# Autodesk Inventor assembly: yaw_unit
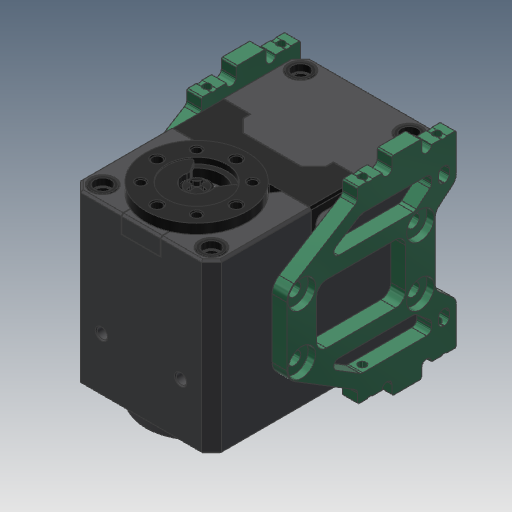
[picture p0: Inventor's stored thumbnail of the model, 512x512]
Saved by Autodesk Inventor 2019.4 (Build 234330000, 330)
## iProperties
Created: 2018-08-06
Part Number: yaw_unit
Material: 一般
Document SubType Name: Assembly
Designer: student
Mass: 66.6076 g
Surface Area: 177.769 cm^2
Volume: 47.0989 cm^3
Density: 1.41421 g/cm^3
Author: student
## Documents named in this file (4)
- C:\Workspace\HaptHexa\Hardware\Inventor\Thorax\yaw_unit\yaw_unit.iam
- C:\Workspace\HaptHexa\Hardware\Inventor\X430\XL-430.iam
- C:\Workspace\HaptHexa\Hardware\Inventor\Thorax\yaw_unit\yaw_servo_side.ipt
- C:\Workspace\HaptHexa\Hardware\Inventor\Thorax\yaw_unit\yaw_servo_side_mir1.ipt
## Components (3 placed, 3 different names)
1. XL-430:1 [sub-assembly] — メイト:1, メイト:2, メイト:3, フラッシュ:1, メイト:4, フラッシュ:2
2. yaw_servo_side:1 — メイト:1, メイト:2, メイト:3
3. yaw_servo_side_mir1:1
## Relationships (6: Mate 4, Flush 2)
- メイト:1 [Mate]: XL-430:1 ↔ yaw_servo_side:1
- メイト:2 [Mate]: XL-430:1 ↔ yaw_servo_side:1
- メイト:3 [Mate]: XL-430:1 ↔ yaw_servo_side:1
- フラッシュ:1 [Flush]: XL-430:1
- メイト:4 [Mate]: XL-430:1
- フラッシュ:2 [Flush]: XL-430:1
